# Autodesk Inventor assembly: mearm組合
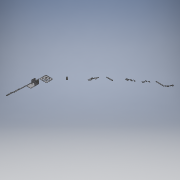
[picture p0: Inventor's stored thumbnail of the model, 180x180]
Saved by Autodesk Inventor 2019 (Build 230136000, 136)
## iProperties
Created: 2022-01-10
Part Number: mearm組合
Material: 一般
Document SubType Name: Assembly
Designer: 10617
Author: 10617
## Documents named in this file (29)
- E:\cad2021\data\tmp\cad2021_hw\downloads\meARM\meARM_Inventor\mearm組合.iam
- E:\cad2021\data\tmp\cad2021_hw\downloads\meARM\meARM_Inventor\mearm零件\1.ipt
- E:\cad2021\data\tmp\cad2021_hw\downloads\meARM\meARM_Inventor\mearm零件\2.ipt
- E:\cad2021\data\tmp\cad2021_hw\downloads\meARM\meARM_Inventor\mearm零件\3.ipt
- E:\cad2021\data\tmp\cad2021_hw\downloads\meARM\meARM_Inventor\mearm零件\4.ipt
- E:\cad2021\data\tmp\cad2021_hw\downloads\meARM\meARM_Inventor\mearm零件\5.ipt
- E:\cad2021\data\tmp\cad2021_hw\downloads\meARM\meARM_Inventor\mearm零件\6.ipt
- E:\cad2021\data\tmp\cad2021_hw\downloads\meARM\meARM_Inventor\mearm零件\7.ipt
- E:\cad2021\data\tmp\cad2021_hw\downloads\meARM\meARM_Inventor\mearm零件\8.ipt
- E:\cad2021\data\tmp\cad2021_hw\downloads\meARM\meARM_Inventor\mearm零件\9.ipt
- E:\cad2021\data\tmp\cad2021_hw\downloads\meARM\meARM_Inventor\mearm零件\10.ipt
- E:\cad2021\data\tmp\cad2021_hw\downloads\meARM\meARM_Inventor\mearm零件\11.ipt
- E:\cad2021\data\tmp\cad2021_hw\downloads\meARM\meARM_Inventor\mearm零件\12.ipt
- E:\cad2021\data\tmp\cad2021_hw\downloads\meARM\meARM_Inventor\mearm零件\13.ipt
- E:\cad2021\data\tmp\cad2021_hw\downloads\meARM\meARM_Inventor\mearm零件\14.ipt
- E:\cad2021\data\tmp\cad2021_hw\downloads\meARM\meARM_Inventor\mearm零件\15.ipt
- E:\cad2021\data\tmp\cad2021_hw\downloads\meARM\meARM_Inventor\mearm零件\16.ipt
- E:\cad2021\data\tmp\cad2021_hw\downloads\meARM\meARM_Inventor\mearm零件\17.ipt
- E:\cad2021\data\tmp\cad2021_hw\downloads\meARM\meARM_Inventor\mearm零件\18.ipt
- E:\cad2021\data\tmp\cad2021_hw\downloads\meARM\meARM_Inventor\mearm零件\19.ipt
- E:\cad2021\data\tmp\cad2021_hw\downloads\meARM\meARM_Inventor\mearm零件\20.ipt
- E:\cad2021\data\tmp\cad2021_hw\downloads\meARM\meARM_Inventor\mearm零件\21.ipt
- E:\cad2021\data\tmp\cad2021_hw\downloads\meARM\meARM_Inventor\mearm零件\22.ipt
- E:\cad2021\data\tmp\cad2021_hw\downloads\meARM\meARM_Inventor\mearm零件\24.ipt
- E:\cad2021\data\tmp\cad2021_hw\downloads\meARM\meARM_Inventor\mearm零件\25.ipt
- E:\cad2021\data\tmp\cad2021_hw\downloads\meARM\meARM_Inventor\mearm零件\26.ipt
- E:\cad2021\data\tmp\cad2021_hw\downloads\meARM\meARM_Inventor\mearm零件\27.ipt
- E:\cad2021\data\tmp\cad2021_hw\downloads\meARM\meARM_Inventor\mearm零件\齒輪.ipt
- E:\cad2021\data\tmp\cad2021_hw\downloads\meARM\meARM_Inventor\mearm零件\齒輪2.ipt
## Components (28 placed, 28 different names)
1. 1:1
2. 2:1
3. 3:1
4. 4:1
5. 5:1
6. 6:1 — 齊平:1, 貼合:1, 貼合:2, 貼合:3, 角度:2, 齊平:3, 角度:3, 齊平:6, 齊平:7
7. 7:1 — 角度:2, 齊平:3, 齊平:4, 齊平:5
8. 8:1 — 貼合:13, 貼合:14, 齊平:9
9. 9:1
10. 10:1 — 貼合:11, 齊平:8, 貼合:12
11. 11:1 — 角度:3, 齊平:6, 齊平:7, 貼合:5, 貼合:6, 貼合:7, 貼合:8, 貼合:9, 貼合:10, 貼合:17, 貼合:19
12. 12:1
13. 13:1
14. 14:1 — 貼合:8, 貼合:9, 貼合:10, 貼合:15, 貼合:16, 齊平:10, 角度:4, 貼合:18
15. 15:1
16. 16:1 — 貼合:5, 貼合:6, 貼合:7, 貼合:11, 齊平:8, 貼合:12, 貼合:13, 貼合:14, 齊平:9
17. 17:1 — 貼合:15, 貼合:16, 齊平:10
18. 18:1
19. 19:1
20. 20:1
21. 21:1 — 貼合:17, 角度:4, 貼合:18, 貼合:19
22. 22:1 — 齊平:1, 貼合:1, 貼合:2, 貼合:3, 齊平:4, 齊平:5
23. 24:1
24. 25:1
25. 26:1
26. 27:1
27. 齒輪:1
28. 齒輪2:1
## Relationships (30: Mate 18, Flush 9, Angle 3)
- 齊平:1 [Flush] (13 mm): 6:1 ↔ 22:1
- 貼合:1 [Mate]: 6:1 ↔ 22:1
- 貼合:2 [Mate]: 6:1 ↔ 22:1
- 貼合:3 [Mate]: 6:1 ↔ 22:1
- 角度:2 [Angle] (0 deg): 6:1 ↔ 7:1
- 齊平:3 [Flush] (-7.63 mm): 6:1 ↔ 7:1
- 齊平:4 [Flush]: 7:1 ↔ 22:1
- 齊平:5 [Flush]: 7:1 ↔ 22:1
- 角度:3 [Angle] (0 deg): 6:1 ↔ 11:1
- 齊平:6 [Flush] (21.31 mm): 6:1 ↔ 11:1
- 齊平:7 [Flush] (-24.48 mm): 6:1 ↔ 11:1
- 貼合:5 [Mate]: 11:1 ↔ 16:1
- 貼合:6 [Mate]: 11:1 ↔ 16:1
- 貼合:7 [Mate]: 11:1 ↔ 16:1
- 貼合:8 [Mate]: 11:1 ↔ 14:1
- 貼合:9 [Mate]: 11:1 ↔ 14:1
- 貼合:10 [Mate]: 11:1 ↔ 14:1
- 貼合:11 [Mate]: 10:1 ↔ 16:1
- 齊平:8 [Flush]: 10:1 ↔ 16:1
- 貼合:12 [Mate]: 10:1 ↔ 16:1
- 貼合:13 [Mate]: 8:1 ↔ 16:1
- 貼合:14 [Mate]: 8:1 ↔ 16:1
- 齊平:9 [Flush] (-5.37 mm): 8:1 ↔ 16:1
- 貼合:15 [Mate]: 14:1 ↔ 17:1
- 貼合:16 [Mate]: 14:1 ↔ 17:1
- 齊平:10 [Flush] (-5.37 mm): 14:1 ↔ 17:1
- 貼合:17 [Mate]: 11:1 ↔ 21:1
- 角度:4 [Angle] (0 deg): 14:1 ↔ 21:1
- 貼合:18 [Mate] (11.88 mm): 14:1 ↔ 21:1
- 貼合:19 [Mate] (3 mm): 11:1 ↔ 21:1
